# Autodesk Inventor assembly: stack_gear_miirrored
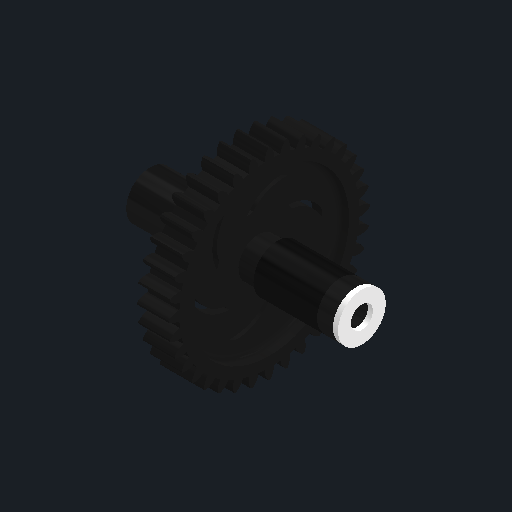
[picture p0: Inventor's stored thumbnail of the model, 512x512]
Saved by Autodesk Inventor 2025 (Build 290162000, 162)
## iProperties
Created: 2024-10-03
Part Number: stack_gear_miirrored
Document SubType Name: Assembly
Designer: Averey Ku
Author: Averey Ku
## Documents named in this file (10)
- D:\vex_robotics_high_stakes\hardware\cad\bots\high_stakes_v2\chassis\drivebay_mirrored\stack_gear_miirrored.iam
- D:\vex_robotics_high_stakes\hardware\cad\bots\high_stakes_v2\chassis\drivebay_mirrored\LS 36T Gear_miirrored.ipt
- D:\vex_robotics_high_stakes\hardware\cad\robpros_cad_lib\Motion\Spacers\Washer Teflon\TWasher .375 OD x .04000.ipt
- D:\vex_robotics_high_stakes\hardware\cad\robpros_cad_lib\Motion\Spacers\Washer Teflon.ipt
- D:\vex_robotics_high_stakes\hardware\cad\robpros_cad_lib\Motion\Spacers\Spacer Nylon .375 OD\NSpacer .375 OD x .500.ipt
- D:\vex_robotics_high_stakes\hardware\cad\robpros_cad_lib\Motion\Spacers\Spacer Nylon .375 OD.ipt
- D:\vex_robotics_high_stakes\hardware\cad\bots\high_stakes_v2\chassis\drivebay_mirrored\Shaft Collar Set Screw_miirrored.ipt
- D:\vex_robotics_high_stakes\hardware\cad\VEX-CAD-Inventor\Motion\Spacers\Spacer Nylon .375 OD\NSpacer .375 OD x .375.ipt
- D:\vex_robotics_high_stakes\hardware\cad\VEX-CAD-Inventor\Motion\Spacers\Spacer Nylon .375 OD.ipt
- D:\vex_robotics_high_stakes\hardware\cad\VEX-CAD-Inventor\Motion\Spacers\Spacer Nylon .375 OD\NSpacer .375 OD x .125.ipt
## Components (6 placed, 6 different names)
1. LS 36T Gear_miirrored:1 — Insert:3, Insert:5
2. TWasher .375 OD x .04000:1 — Insert:8
3. NSpacer .375 OD x .500:1 — Insert:3, Insert:7
4. Shaft Collar Set Screw_miirrored:1 — Insert:5, Insert:6
5. NSpacer .375 OD x .375:2 — Insert:6
6. NSpacer .375 OD x .125:3 — Insert:8, Insert:7
## Relationships (5: Insert 5)
- Insert:3: LS 36T Gear_miirrored:1 ↔ NSpacer .375 OD x .500:1
- Insert:5: LS 36T Gear_miirrored:1 ↔ Shaft Collar Set Screw_miirrored:1
- Insert:6: Shaft Collar Set Screw_miirrored:1 ↔ NSpacer .375 OD x .375:2
- Insert:8: TWasher .375 OD x .04000:1 ↔ NSpacer .375 OD x .125:3
- Insert:7: NSpacer .375 OD x .500:1 ↔ NSpacer .375 OD x .125:3
